# Autodesk Inventor assembly: 50
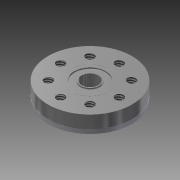
[picture p0: Inventor's stored thumbnail of the model, 180x180]
Saved by Autodesk Inventor 2013 (Build 170138000, 138)
## iProperties
Created: 2014-03-12
Part Number: 50
Document SubType Name: Assembly
Designer: andou
Mass: 3.41694 g
Surface Area: 18.585 cm^2
Volume: 1.11522 cm^3
Density: 3.06393 g/cm^3
Author: andou
Title: Free_Horn
## Documents named in this file (5)
- C:\Users\andou\Documents\Inventor\RoboticsProject\project_4\Robot\Free_Horn\Free_Horn.iam
- C:\Users\andou\Documents\Inventor\RoboticsProject\project_4\Robot\Free_Horn\Bearing Holder.ipt
- C:\Users\andou\Documents\Inventor\RoboticsProject\project_4\Robot\Free_Horn\Bearing.ipt
- C:\Users\andou\Documents\Inventor\RoboticsProject\project_4\Robot\Free_Horn\Acetal_Washer(t1.0).ipt
- C:\Users\andou\Documents\Inventor\RoboticsProject\project_4\Robot\Free_Horn\Bearing_Washer(t1.0).ipt
## Components (4 placed, 4 different names)
1. Bearing Holder:1 — 挿入:1, 挿入:2, 挿入:4
2. Bearing:1 — 挿入:1, 挿入:3, 挿入:4
3. Acetal_Washer(t1.0):1 — 挿入:2
4. Bearing_Washer(t1.0):1 — 挿入:3
## Relationships (4: Insert 4)
- 挿入:1 [Insert]: Bearing Holder:1 ↔ Bearing:1
- 挿入:2 [Insert]: Bearing Holder:1 ↔ Acetal_Washer(t1.0):1
- 挿入:3 [Insert]: Bearing:1 ↔ Bearing_Washer(t1.0):1
- 挿入:4 [Insert]: Bearing Holder:1 ↔ Bearing:1
